# Autodesk Inventor assembly: IV Stand STEP
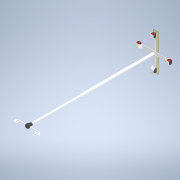
[picture p0: Inventor's stored thumbnail of the model, 180x180]
Saved by Autodesk Inventor 2020.3 (Build 243373000, 373)
## iProperties
Created: 2014-12-03
Part Number: IV Stand STEP
Description: STEP AP214
Document SubType Name: Assembly
Designer: Bruno
Preprocessor: Spatial InterOp 3D
Title: IV Stand STEP.stp
Revision Number: NONE
## Documents named in this file (5)
- C:\Users\Bruno\Desktop\CNAF\CNAF-3\IV Stand Medical\IV Stand STEP.iam
- C:\Users\Bruno\Desktop\CNAF\CNAF-3\IV Stand Medical\Assembly129.iam
- C:\Users\Bruno\Desktop\CNAF\CNAF-3\IV Stand Medical\Assembly129_1.iam
- C:\Users\Bruno\Desktop\CNAF\CNAF-3\IV Stand Medical\Part133.ipt
- C:\Users\Bruno\Desktop\CNAF\CNAF-3\IV Stand Medical\Part137.ipt
## Components (4 placed, 3 different names)
1. Assembly129 [sub-assembly]
2. Assembly129:1 [sub-assembly] — Angle:1, Tangent:1
3. Part133
4. Part137
## Relationships (2: Angle 1, Tangent 1)
- Angle:1 (0 deg): Assembly129:1
- Tangent:1: Assembly129:1
